# Autodesk Inventor assembly: 3_left_leg_true_final
(part 3 of 3)
73. M2x6 Bolt:13 — Rigid:60
74. M2x6 Bolt:14 — Rigid:61
75. M2x6 Bolt:15 — Rigid:62
76. M2x6 Bolt:16 — Rigid:63
77. M2x6 Bolt:17 — Rigid:64
78. M2x6 Bolt:18 — Rigid:65
79. M2x6 Bolt:19 — Rigid:66
80. M2x6 Bolt:20 — Rigid:67
81. M2x6 Bolt:21 — Rigid:68
82. M2x6 Bolt:22 — Rigid:69
83. M2x6 Bolt:23 — Rigid:70
84. M2x6 Bolt:24 — Rigid:71
85. M2x6 Bolt:25 — Rigid:72
86. M2x6 Bolt:26 — Rigid:73
87. M2x6 Bolt:27 — Rigid:74
88. M2x6 Bolt:28 — Rigid:75
89. M2x6 Bolt:29 — Rigid:76
90. M2x6 Bolt:30 — Rigid:77
91. M2x6 Bolt:31 — Rigid:78
92. M2x6 Bolt:32 — Rigid:79
93. M2x6 Bolt:33 — Rigid:83
94. M2x6 Bolt:34 — Rigid:80
95. M2x6 Bolt:35 — Rigid:81
96. M2x6 Bolt:36 — Rigid:82
97. M2x6 Bolt:37 — Rigid:84
98. M2x6 Bolt:38 — Rigid:85
99. M2x6 Bolt:39 — Rigid:86
100. M2x6 Bolt:40 — Rigid:87
101. M3x6 Bolt:1 — Rigid:33
102. M3x6 Bolt:2 — Rigid:32
103. M3x6 Bolt:3 — Rigid:34
104. M3x6 Bolt:4 — Rigid:35
105. M3x6 Bolt:5 — Rigid:36
106. M3x6 Bolt:6 — Rigid:37
107. M3x6 Bolt:7 — Rigid:38
108. M3x6 Bolt:8 — Rigid:39
109. M3 Nut:1 — Rigid:40
110. M3 Nut:2 — Rigid:41
111. M3 Nut:3 — Rigid:42
112. M3 Nut:4 — Rigid:43
113. M3 Nut:5 — Rigid:44
114. M3 Nut:6 — Rigid:45
115. M3 Nut:7 — Rigid:46
116. M3 Nut:8 — Rigid:47
117. M5x10 Bolt:4 — Rigid:28
118. M5 Nylon Nut:1 — Rigid:29
119. M5 Nylon Nut:2 — Rigid:31
120. M5x10 Bolt:1 — Rigid:30
## Relationships (120: WeldJoint 112, RevoluteJoint 8)
- Rotational:1 [RevoluteJoint]: Top Horn:1 ↔ HTD-45H:1
- Rigid:1 [WeldJoint]: axis_1_top_frame:1 ↔ Top Horn:1
- Rotational:2 [RevoluteJoint]: Top Horn:2 ↔ HTD-45H:2
- Rigid:2 [WeldJoint]: axis_1_top_frame:1 ↔ Top Horn:2
- Rotational:3 [RevoluteJoint]: HTD-45H:3 ↔ Top Horn:3
- Rigid:5 [WeldJoint]: axis_1_supplement_frame:1 ↔ axis_1_top_frame:1
- Rigid:7 [WeldJoint]: axis_2_4_connector_frame_powered:1 ↔ Top Horn:3
- Rigid:8 [WeldJoint]: axis_2_4_connector_frame_non_powered:1 ↔ Bottom Horn:3
- Rotational:5 [RevoluteJoint]: Top Horn:4 ↔ HTD-45H:4
- Rigid:11 [WeldJoint]: HTD-45H:4 ↔ 3D_printed_part_powered:1
- Rigid:12 [WeldJoint]: Top Horn:4 ↔ axis_4_5_connector_frame_powered:1
- Rigid:13 [WeldJoint]: Bottom Horn:4 ↔ axis_4_5_connector_frame_non_powered:1
- Rotational:7 [RevoluteJoint]: HTD-45H:5 ↔ Top Horn:5
- Rotational:8 [RevoluteJoint]: HTD-45H:5 ↔ Bottom Horn:5
- Rigid:14 [WeldJoint]: HTD-45H:5 ↔ axis_5_top_frame:1
- Rigid:16 [WeldJoint]: HTD-45H:6 ↔ axis_6_top_frame:1
- Rotational:9 [RevoluteJoint]: Top Horn:6 ↔ HTD-45H:6
- Rigid:17 [WeldJoint]: axis_5_top_frame:1 ↔ axis_6_top_frame:1
- Rigid:18 [WeldJoint]: axis_6_bottom_frame(top):1 ↔ axis_6_supplement_frame:1
- Rigid:19 [WeldJoint]: Top Horn:6 ↔ axis_6_bottom_frame(top):1
- Rigid:20 [WeldJoint]: axis_6_bottom_frame(top):1 ↔ axis_6_bottom_frame(bottom):1
- Rigid:21 [WeldJoint]: HTD-45H:4 ↔ 3D_printed_part_non_powered:1
- Rigid:22 [WeldJoint]: axis_4_5_connector_frame_non_powered:1 ↔ Bottom Horn:5
- Rigid:23 [WeldJoint]: axis_2_4_connector_frame_powered:1 ↔ 3D_printed_part_powered:1
- Rigid:24 [WeldJoint]: axis_2_4_connector_frame_non_powered:1 ↔ 3D_printed_part_non_powered:1
- Rigid:25 [WeldJoint]: axis_2_bottom_frame:1 ↔ HTD-45H:3
- Rigid:26 [WeldJoint]: axis_3_bottom_frame:1 ↔ HTD-45H:2
- Rigid:27 [WeldJoint]: axis_2_bottom_frame:1 ↔ axis_3_bottom_frame:1
- Rigid:28 [WeldJoint]: axis_1_supplement_frame:1 ↔ M5x10 Bolt:4
- Rigid:29 [WeldJoint]: axis_1_top_frame:1 ↔ M5 Nylon Nut:1
- Rigid:30 [WeldJoint]: axis_6_supplement_frame:1 ↔ M5x10 Bolt:1
- Rigid:31 [WeldJoint]: axis_6_bottom_frame(top):1 ↔ M5 Nylon Nut:2
- Rigid:32 [WeldJoint]: axis_6_top_frame:1 ↔ M3x6 Bolt:2
- Rigid:33 [WeldJoint]: axis_6_top_frame:1 ↔ M3x6 Bolt:1
- Rigid:34 [WeldJoint]: axis_6_top_frame:1 ↔ M3x6 Bolt:3
- Rigid:35 [WeldJoint]: axis_6_top_frame:1 ↔ M3x6 Bolt:4
- Rigid:36 [WeldJoint]: axis_2_bottom_frame:1 ↔ M3x6 Bolt:5
- Rigid:37 [WeldJoint]: axis_2_bottom_frame:1 ↔ M3x6 Bolt:6
- Rigid:38 [WeldJoint]: axis_2_bottom_frame:1 ↔ M3x6 Bolt:7
- Rigid:39 [WeldJoint]: axis_2_bottom_frame:1 ↔ M3x6 Bolt:8
- Rigid:40 [WeldJoint]: axis_5_top_frame:1 ↔ M3 Nut:1
- Rigid:41 [WeldJoint]: axis_5_top_frame:1 ↔ M3 Nut:2
- Rigid:42 [WeldJoint]: axis_5_top_frame:1 ↔ M3 Nut:3
- Rigid:43 [WeldJoint]: axis_5_top_frame:1 ↔ M3 Nut:4
- Rigid:44 [WeldJoint]: axis_3_bottom_frame:1 ↔ M3 Nut:5
- Rigid:45 [WeldJoint]: axis_3_bottom_frame:1 ↔ M3 Nut:6
- Rigid:46 [WeldJoint]: axis_3_bottom_frame:1 ↔ M3 Nut:7
- Rigid:47 [WeldJoint]: axis_3_bottom_frame:1 ↔ M3 Nut:8
- Rigid:48 [WeldJoint]: axis_5_top_frame:1 ↔ M2x6 Bolt:1
- Rigid:49 [WeldJoint]: axis_5_top_frame:1 ↔ M2x6 Bolt:2
- Rigid:50 [WeldJoint]: axis_5_top_frame:1 ↔ M2x6 Bolt:3
- Rigid:51 [WeldJoint]: axis_5_top_frame:1 ↔ M2x6 Bolt:4
- Rigid:52 [WeldJoint]: axis_5_top_frame:1 ↔ M2x6 Bolt:5
- Rigid:53 [WeldJoint]: axis_5_top_frame:1 ↔ M2x6 Bolt:6
- Rigid:54 [WeldJoint]: axis_5_top_frame:1 ↔ M2x6 Bolt:7
- Rigid:55 [WeldJoint]: axis_5_top_frame:1 ↔ M2x6 Bolt:8
- Rigid:56 [WeldJoint]: axis_5_top_frame:1 ↔ M2x6 Bolt:9
- Rigid:57 [WeldJoint]: axis_6_top_frame:1 ↔ M2x6 Bolt:10
- Rigid:58 [WeldJoint]: axis_6_top_frame:1 ↔ M2x6 Bolt:11
- Rigid:59 [WeldJoint]: axis_6_top_frame:1 ↔ M2x6 Bolt:12
- Rigid:60 [WeldJoint]: axis_6_top_frame:1 ↔ M2x6 Bolt:13
- Rigid:61 [WeldJoint]: axis_6_top_frame:1 ↔ M2x6 Bolt:14
- Rigid:62 [WeldJoint]: axis_2_bottom_frame:1 ↔ M2x6 Bolt:15
- Rigid:63 [WeldJoint]: axis_2_bottom_frame:1 ↔ M2x6 Bolt:16
- Rigid:64 [WeldJoint]: axis_2_bottom_frame:1 ↔ M2x6 Bolt:17
- Rigid:65 [WeldJoint]: axis_2_bottom_frame:1 ↔ M2x6 Bolt:18
- Rigid:66 [WeldJoint]: axis_2_bottom_frame:1 ↔ M2x6 Bolt:19
- Rigid:67 [WeldJoint]: axis_2_bottom_frame:1 ↔ M2x6 Bolt:20
- Rigid:68 [WeldJoint]: axis_2_bottom_frame:1 ↔ M2x6 Bolt:21
- Rigid:69 [WeldJoint]: axis_2_bottom_frame:1 ↔ M2x6 Bolt:22
- Rigid:70 [WeldJoint]: axis_2_bottom_frame:1 ↔ M2x6 Bolt:23
- Rigid:71 [WeldJoint]: axis_3_bottom_frame:1 ↔ M2x6 Bolt:24
- Rigid:72 [WeldJoint]: axis_3_bottom_frame:1 ↔ M2x6 Bolt:25
- Rigid:73 [WeldJoint]: axis_3_bottom_frame:1 ↔ M2x6 Bolt:26
- Rigid:74 [WeldJoint]: axis_3_bottom_frame:1 ↔ M2x6 Bolt:27
- Rigid:75 [WeldJoint]: axis_3_bottom_frame:1 ↔ M2x6 Bolt:28
- Rigid:76 [WeldJoint]: axis_6_supplement_frame:1 ↔ M2x6 Bolt:29
- Rigid:77 [WeldJoint]: axis_6_supplement_frame:1 ↔ M2x6 Bolt:30
- Rigid:78 [WeldJoint]: axis_6_supplement_frame:1 ↔ M2x6 Bolt:31
- Rigid:79 [WeldJoint]: axis_6_supplement_frame:1 ↔ M2x6 Bolt:32
- Rigid:83 [WeldJoint]: axis_1_supplement_frame:1 ↔ M2x6 Bolt:33
- Rigid:80 [WeldJoint]: axis_1_supplement_frame:1 ↔ M2x6 Bolt:34
- Rigid:81 [WeldJoint]: axis_1_supplement_frame:1 ↔ M2x6 Bolt:35
- Rigid:82 [WeldJoint]: axis_1_supplement_frame:1 ↔ M2x6 Bolt:36
- Rigid:84 [WeldJoint]: axis_1_supplement_frame:1 ↔ M2x6 Bolt:37
- Rigid:85 [WeldJoint]: axis_1_supplement_frame:1 ↔ M2x6 Bolt:38
- Rigid:86 [WeldJoint]: axis_1_supplement_frame:1 ↔ M2x6 Bolt:39
- Rigid:87 [WeldJoint]: axis_1_supplement_frame:1 ↔ M2x6 Bolt:40
- Rigid:88 [WeldJoint]: axis_4_5_connector_frame_powered:1 ↔ M2x4 Bolt:1
- Rigid:89 [WeldJoint]: axis_4_5_connector_frame_powered:1 ↔ M2x4 Bolt:2
- Rigid:90 [WeldJoint]: axis_4_5_connector_frame_powered:1 ↔ M2x4 Bolt:3
- Rigid:91 [WeldJoint]: axis_4_5_connector_frame_powered:1 ↔ M2x4 Bolt:4
- Rigid:92 [WeldJoint]: axis_4_5_connector_frame_powered:1 ↔ M2x4 Bolt:5
- Rigid:93 [WeldJoint]: axis_4_5_connector_frame_powered:1 ↔ M2x4 Bolt:6
- Rigid:94 [WeldJoint]: axis_4_5_connector_frame_powered:1 ↔ M2x4 Bolt:7
- Rigid:95 [WeldJoint]: axis_4_5_connector_frame_powered:1 ↔ M2x4 Bolt:8
- Rigid:96 [WeldJoint]: axis_2_4_connector_frame_powered:1 ↔ M2x4 Bolt:9
- Rigid:97 [WeldJoint]: axis_2_4_connector_frame_powered:1 ↔ M2x4 Bolt:10
- Rigid:98 [WeldJoint]: axis_2_4_connector_frame_powered:1 ↔ M2x4 Bolt:11
- Rigid:99 [WeldJoint]: axis_2_4_connector_frame_powered:1 ↔ M2x4 Bolt:12
- Rigid:100 [WeldJoint]: axis_4_5_connector_frame_non_powered:1 ↔ M2x4 Bolt:13
- Rigid:101 [WeldJoint]: axis_4_5_connector_frame_non_powered:1 ↔ M2x4 Bolt:14
- Rigid:102 [WeldJoint]: axis_4_5_connector_frame_non_powered:1 ↔ M2x4 Bolt:15
- Rigid:103 [WeldJoint]: axis_4_5_connector_frame_non_powered:1 ↔ M2x4 Bolt:16
- Rigid:104 [WeldJoint]: axis_4_5_connector_frame_non_powered:1 ↔ M2x4 Bolt:17
- Rigid:105 [WeldJoint]: axis_4_5_connector_frame_non_powered:1 ↔ M2x4 Bolt:18
- Rigid:106 [WeldJoint]: axis_4_5_connector_frame_non_powered:1 ↔ M2x4 Bolt:19
- Rigid:107 [WeldJoint]: axis_4_5_connector_frame_non_powered:1 ↔ M2x4 Bolt:20
- Rigid:108 [WeldJoint]: axis_2_4_connector_frame_non_powered:1 ↔ M2x4 Bolt:21
- Rigid:109 [WeldJoint]: axis_2_4_connector_frame_non_powered:1 ↔ M2x4 Bolt:22
- Rigid:110 [WeldJoint]: axis_2_4_connector_frame_non_powered:1 ↔ M2x4 Bolt:23
- Rigid:111 [WeldJoint]: axis_2_4_connector_frame_non_powered:1 ↔ M2x4 Bolt:24
- Rotational:113 [RevoluteJoint]: Bottom Horn:4 ↔ HTD-45H:4
- Rigid:112 [WeldJoint]: axis_4_5_connector_frame_powered:1 ↔ Top Horn:5
- Rigid:113 [WeldJoint]: M2x12 Bolt:1 ↔ axis_2_4_connector_frame_powered:1
- Rigid:114 [WeldJoint]: M2x12 Bolt:2 ↔ axis_2_4_connector_frame_powered:1
- Rigid:115 [WeldJoint]: M2x12 Bolt:3 ↔ axis_2_4_connector_frame_powered:1
- Rigid:116 [WeldJoint]: M2x12 Bolt:4 ↔ axis_2_4_connector_frame_non_powered:1
- Rigid:117 [WeldJoint]: M2x12 Bolt:5 ↔ axis_2_4_connector_frame_non_powered:1
- Rigid:118 [WeldJoint]: M2x12 Bolt:6 ↔ axis_2_4_connector_frame_non_powered:1
